# Autodesk Inventor assembly: matt, double drive
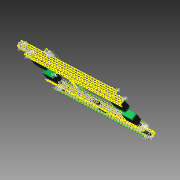
[picture p0: Inventor's stored thumbnail of the model, 180x180]
Saved by Autodesk Inventor 2014 (Build 180170000, 170)
## iProperties
Created: 2014-08-19
Part Number: matt, double drive
Document SubType Name: Assembly
Designer: Josef
Author: Josef
## Documents named in this file (5)
- C:\Users\Josef\Documents\Vex parts\#1 sub assemblys\Drive\matt, double drive.iam
- C:\Users\Josef\Documents\Vex parts\Metal C-Channels\Aluminum C-Channel 1x2x1x35.ipt
- C:\Users\Josef\Documents\Vex parts\Bearingw-screws.iam
- C:\Users\Josef\Documents\Vex parts\Metal C-Channels\Aluminum C-Channel 1x2x1x21.ipt
- C:\Users\Josef\Documents\Vex parts\motor w-screw.iam
## Components (13 placed, 4 different names)
1. Aluminum C-Channel 1x2x1x35:1 — Mate:2, Mate:3, Mate:6, Mate:7, Mate:8, Mate:11, Mate:12, Mate:15, Mate:16, Flush:1, Flush:3, Flush:4
2. Aluminum C-Channel 1x2x1x35:2 — Mate:4, Mate:17, Mate:18, Mate:19, Flush:1, Flush:2, Flush:3, Flush:5, Flush:12, Mate:29, Mate:30, Mate:31, Mate:32
3. Bearingw-screws:2 [sub-assembly] — Mate:4, Mate:17, Mate:18
4. Bearingw-screws:4 [sub-assembly] — Mate:2, Mate:7, Mate:8, Mate:33, Mate:34
5. Bearingw-screws:5 [sub-assembly] — Mate:3, Mate:15, Mate:16
6. Bearingw-screws:6 [sub-assembly] — Mate:6, Mate:11, Mate:12
7. Aluminum C-Channel 1x2x1x21:1 — Mate:19, Flush:2, Flush:4, Flush:5, Mate:20, Flush:10, Flush:11
8. Aluminum C-Channel 1x2x1x35:3 — Flush:6, Flush:9, Flush:10
9. Aluminum C-Channel 1x2x1x35:4 — Mate:20, Flush:6, Flush:9, Flush:11, Flush:12, Mate:21, Mate:22, Mate:23, Mate:24, Mate:25, Mate:26, Mate:27, Mate:28
10. motor w-screw:1 [sub-assembly] — Mate:21, Mate:22, Mate:23, Mate:24
11. motor w-screw:2 [sub-assembly] — Mate:25, Mate:26, Mate:27, Mate:28
12. motor w-screw:3 [sub-assembly] — Mate:32, Mate:33, Mate:34
13. motor w-screw:4 [sub-assembly] — Mate:29, Mate:30, Mate:31
## Relationships (38: Mate 28, Flush 10)
- Mate:2: Aluminum C-Channel 1x2x1x35:1 ↔ Bearingw-screws:4
- Mate:3: Aluminum C-Channel 1x2x1x35:1 ↔ Bearingw-screws:5
- Mate:4: Aluminum C-Channel 1x2x1x35:2 ↔ Bearingw-screws:2
- Mate:6: Aluminum C-Channel 1x2x1x35:1 ↔ Bearingw-screws:6
- Mate:7: Aluminum C-Channel 1x2x1x35:1 ↔ Bearingw-screws:4
- Mate:8: Aluminum C-Channel 1x2x1x35:1 ↔ Bearingw-screws:4
- Mate:11: Aluminum C-Channel 1x2x1x35:1 ↔ Bearingw-screws:6
- Mate:12: Aluminum C-Channel 1x2x1x35:1 ↔ Bearingw-screws:6
- Mate:15: Aluminum C-Channel 1x2x1x35:1 ↔ Bearingw-screws:5
- Mate:16: Aluminum C-Channel 1x2x1x35:1 ↔ Bearingw-screws:5
- Mate:17: Aluminum C-Channel 1x2x1x35:2 ↔ Bearingw-screws:2
- Mate:18: Aluminum C-Channel 1x2x1x35:2 ↔ Bearingw-screws:2
- Mate:19: Aluminum C-Channel 1x2x1x35:2 ↔ Aluminum C-Channel 1x2x1x21:1
- Flush:1: Aluminum C-Channel 1x2x1x35:1 ↔ Aluminum C-Channel 1x2x1x35:2
- Flush:2: Aluminum C-Channel 1x2x1x35:2 ↔ Aluminum C-Channel 1x2x1x21:1
- Flush:3: Aluminum C-Channel 1x2x1x35:1 ↔ Aluminum C-Channel 1x2x1x35:2
- Flush:4: Aluminum C-Channel 1x2x1x35:1 ↔ Aluminum C-Channel 1x2x1x21:1
- Flush:5: Aluminum C-Channel 1x2x1x35:2 ↔ Aluminum C-Channel 1x2x1x21:1
- Mate:20: Aluminum C-Channel 1x2x1x21:1 ↔ Aluminum C-Channel 1x2x1x35:4
- Flush:6: Aluminum C-Channel 1x2x1x35:3 ↔ Aluminum C-Channel 1x2x1x35:4
- Flush:9: Aluminum C-Channel 1x2x1x35:3 ↔ Aluminum C-Channel 1x2x1x35:4
- Flush:10: Aluminum C-Channel 1x2x1x21:1 ↔ Aluminum C-Channel 1x2x1x35:3
- Flush:11: Aluminum C-Channel 1x2x1x21:1 ↔ Aluminum C-Channel 1x2x1x35:4
- Flush:12: Aluminum C-Channel 1x2x1x35:2 ↔ Aluminum C-Channel 1x2x1x35:4
- Mate:21: Aluminum C-Channel 1x2x1x35:4 ↔ motor w-screw:1
- Mate:22: Aluminum C-Channel 1x2x1x35:4 ↔ motor w-screw:1
- Mate:23: Aluminum C-Channel 1x2x1x35:4 ↔ motor w-screw:1
- Mate:24: Aluminum C-Channel 1x2x1x35:4 ↔ motor w-screw:1
- Mate:25: Aluminum C-Channel 1x2x1x35:4 ↔ motor w-screw:2
- Mate:26: Aluminum C-Channel 1x2x1x35:4 ↔ motor w-screw:2
- Mate:27: Aluminum C-Channel 1x2x1x35:4 ↔ motor w-screw:2
- Mate:28: Aluminum C-Channel 1x2x1x35:4 ↔ motor w-screw:2
- Mate:29: Aluminum C-Channel 1x2x1x35:2 ↔ motor w-screw:4
- Mate:30: Aluminum C-Channel 1x2x1x35:2 ↔ motor w-screw:4
- Mate:31: Aluminum C-Channel 1x2x1x35:2 ↔ motor w-screw:4
- Mate:32: Aluminum C-Channel 1x2x1x35:2 ↔ motor w-screw:3
- Mate:33: Bearingw-screws:4 ↔ motor w-screw:3
- Mate:34: Bearingw-screws:4 ↔ motor w-screw:3
